# Autodesk Inventor assembly: Assembly1
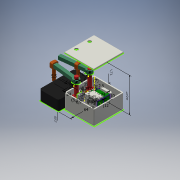
[picture p0: Inventor's stored thumbnail of the model, 180x180]
Saved by Autodesk Inventor 2019 (Build 230136000, 136)
## iProperties
Created: 2020-07-23
Part Number: Assembly1
Document SubType Name: Assembly
Designer: lukad
Author: lukad
## Documents named in this file (14)
- D:\KEYBOT\Assembly1.iam
- D:\KEYBOT\ohisje.ipt
- D:\KEYBOT\ohisje_pokrov.ipt
- D:\KEYBOT\pin.ipt
- D:\KEYBOT\kolo.ipt
- D:\KEYBOT\VZMET4mm.ipt
- D:\KEYBOT\vzmetzgoraj.ipt
- D:\KEYBOT\motorcek.ipt
- D:\KEYBOT\baterija.ipt
- D:\KEYBOT\roka1.ipt
- D:\KEYBOT\roka2.ipt
- D:\KEYBOT\kluc.ipt
- D:\KEYBOT\čip.ipt
- D:\KEYBOT\koncnostikalo.ipt
## Components (18 placed, 13 different names)
1. ohisje:1 — Mate:1, Mate:2, Cylindrical:1, Cylindrical:2, Rotational:1, Mate:15, Rigid:1, Rigid:2, Slider:1, Slider:2, Mate:22, Flush:1, Mate:23, Mate:24, Mate:25, Mate:26, Mate:27, Mate:28, Flush:2
2. ohisje_pokrov:1 — Mate:1, Mate:2, Mate:15, Mate:16, Mate:17, Mate:18, Mate:19
3. pin:2 — Slider:1, Cylindrical:4
4. kolo:1 — Cylindrical:1, Cylindrical:2, Rotational:1, Mate:20, Mate:21
5. pin:3 — Slider:2, Cylindrical:3
6. VZMET4mm:2 — Rigid:2
7. VZMET4mm:3 — Rigid:1
8. vzmetzgoraj:1 — Mate:18, Mate:19
9. vzmetzgoraj:2 — Mate:16, Mate:17
10. motorcek:1 — Mate:20, Mate:21, Mate:22, Flush:1
11. baterija:2 — Mate:23
12. roka1:1 — Cylindrical:3, Slider:3
13. roka2:1 — Slider:3
14. kluc:1 — Mate:24, Mate:25
15. roka1:2 — Cylindrical:4, Slider:4
16. roka2:2 — Slider:4
17. čip:1 — Mate:26, Mate:27
18. koncnostikalo:1 — Mate:28, Flush:2
## Relationships (29: Mate 16, CylindricalJoint 4, TranslationJoint 4, WeldJoint 2, Flush 2, RevoluteJoint 1)
- Mate:1: ohisje:1 ↔ ohisje_pokrov:1
- Mate:2: ohisje:1 ↔ ohisje_pokrov:1
- Cylindrical:1: ohisje:1 ↔ kolo:1
- Cylindrical:2: ohisje:1 ↔ kolo:1
- Rotational:1 [RevoluteJoint]: ohisje:1 ↔ kolo:1
- Mate:15: ohisje:1 ↔ ohisje_pokrov:1
- Rigid:1 [WeldJoint]: ohisje:1 ↔ VZMET4mm:3
- Rigid:2 [WeldJoint]: ohisje:1 ↔ VZMET4mm:2
- Slider:1 [TranslationJoint]: ohisje:1 ↔ pin:2
- Mate:16: ohisje_pokrov:1 ↔ vzmetzgoraj:2
- Mate:17 (-0.25 mm): ohisje_pokrov:1 ↔ vzmetzgoraj:2
- Mate:18: ohisje_pokrov:1 ↔ vzmetzgoraj:1
- Mate:19 (-0.25 mm): ohisje_pokrov:1 ↔ vzmetzgoraj:1
- Slider:2 [TranslationJoint]: ohisje:1 ↔ pin:3
- Mate:20: kolo:1 ↔ motorcek:1
- Mate:21 (0.3 mm): kolo:1 ↔ motorcek:1
- Mate:22: ohisje:1 ↔ motorcek:1
- Flush:1: ohisje:1 ↔ motorcek:1
- Mate:23: ohisje:1 ↔ baterija:2
- Cylindrical:3: pin:3 ↔ roka1:1
- Slider:3 [TranslationJoint]: roka1:1 ↔ roka2:1
- Mate:24: ohisje:1 ↔ kluc:1
- Mate:25: ohisje:1 ↔ kluc:1
- Cylindrical:4: pin:2 ↔ roka1:2
- Slider:4 [TranslationJoint]: roka1:2 ↔ roka2:2
- Mate:26: ohisje:1 ↔ čip:1
- Mate:27: ohisje:1 ↔ čip:1
- Mate:28: ohisje:1 ↔ koncnostikalo:1
- Flush:2: ohisje:1 ↔ koncnostikalo:1
